# Autodesk Inventor assembly: Ass eyebrow
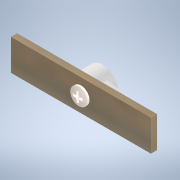
[picture p0: Inventor's stored thumbnail of the model, 180x180]
Saved by Autodesk Inventor 2021 (Build 250183000, 183)
## iProperties
Created: 2023-06-07
Part Number: Ass eyebrow
Document SubType Name: Assembly
Designer: shrus
Author: shrus
## Documents named in this file (4)
- C:\Users\shrus\Documents\Ass eyebrow.iam
- C:\Users\shrus\Documents\Moving eyebrow2.ipt
- C:\Users\shrus\Documents\servoarm1.ipt
- C:\Users\shrus\Documents\m3-5mm.ipt
## Components (3 placed, 3 different names)
1. Moving eyebrow2:1 — Mate:1, Mate:2, Mate:3
2. servoarm1:1 — Mate:1, Mate:2
3. m3-5mm:1 — Mate:3
## Relationships (3: Mate 3)
- Mate:1: Moving eyebrow2:1 ↔ servoarm1:1
- Mate:2: Moving eyebrow2:1 ↔ servoarm1:1
- Mate:3: Moving eyebrow2:1 ↔ m3-5mm:1
